# Autodesk Inventor assembly: Neck_assembly001
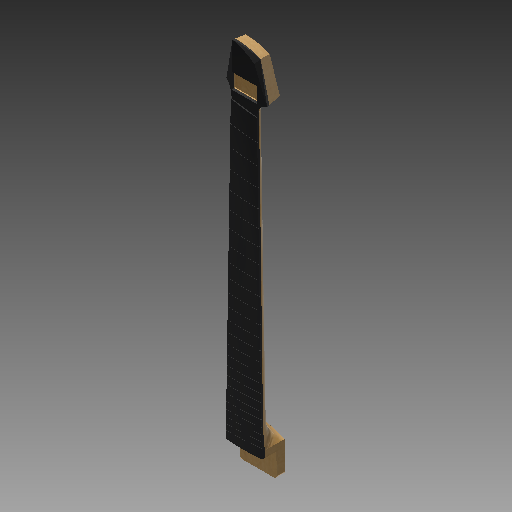
[picture p0: Inventor's stored thumbnail of the model, 512x512]
Saved by Autodesk Inventor 2017 (Build 210142000, 142)
## iProperties
Created: 2016-06-14
Part Number: Neck_assembly001
Document SubType Name: Assembly
Designer: Andy
Author: Andy
## Documents named in this file (3)
- C:\Users\Andy\Desktop\CAD\Guitar\Compass\Neck_assembly001.iam
- C:\Users\Andy\Desktop\CAD\Guitar\Compass\Neck001.ipt
- C:\Users\Andy\Desktop\CAD\Guitar\Compass\Fret_Board001.ipt
## Components (2 placed, 2 different names)
1. Neck001:1 — Mate:1, Mate:2
2. Fret_Board001:1 — Mate:1, Mate:2
## Relationships (2: Mate 2)
- Mate:1: Neck001:1 ↔ Fret_Board001:1
- Mate:2: Neck001:1 ↔ Fret_Board001:1
